# Autodesk Inventor assembly: claw
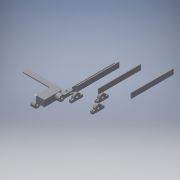
[picture p0: Inventor's stored thumbnail of the model, 180x180]
Saved by Autodesk Inventor 2017 (Build 210142000, 142)
## iProperties
Created: 2017-04-28
Part Number: claw
Document SubType Name: Assembly
Designer: s4321966
Author: s4321966
## Documents named in this file (5)
- \\puffball.labs.eait.uq.edu.au\s4321966\Documents\metr4810_spool draft\claw.iam
- \\puffball.labs.eait.uq.edu.au\s4321966\Documents\metr4810_spool draft\attachment.ipt
- \\puffball.labs.eait.uq.edu.au\s4321966\Documents\metr4810_spool draft\bar.ipt
- \\puffball.labs.eait.uq.edu.au\s4321966\Documents\metr4810_spool draft\servo attachment.ipt
- \\puffball.labs.eait.uq.edu.au\s4321966\Documents\metr4810_spool draft\servo.ipt
## Components (12 placed, 4 different names)
1. attachment:1
2. bar:1 — Flush:1, Mate:2, Flush:2
3. servo attachment:1 — Mate:1, Tangent:1, Flush:1, Mate:2, Flush:2
4. servo:1 — Mate:1, Tangent:1
5. attachment:2
6. attachment:3
7. servo attachment:2
8. bar:2
9. bar:3
10. bar:4
11. bar:5
12. bar:6
## Relationships (5: Mate 2, Flush 2, Tangent 1)
- Mate:1: servo attachment:1 ↔ servo:1
- Tangent:1: servo attachment:1 ↔ servo:1
- Flush:1: bar:1 ↔ servo attachment:1
- Mate:2: bar:1 ↔ servo attachment:1
- Flush:2: bar:1 ↔ servo attachment:1
